# Autodesk Inventor assembly: ASY ДМФ 0100 Барабан v2.1
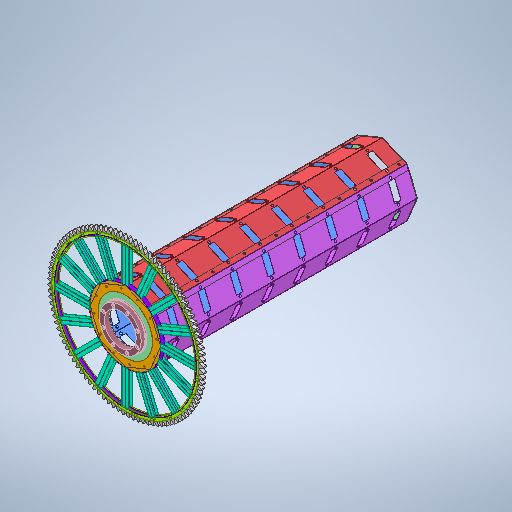
[picture p0: Inventor's stored thumbnail of the model, 512x512]
Saved by Autodesk Inventor 2025 (Build 290162010, 162A)
## iProperties
Created: 2024-04-28
Part Number: ASY ДМФ 0100 Барабан v2.1
Document SubType Name: Assembly
Designer: pokla
Author: pokla
## Documents named in this file (20)
- C:\Users\pokla\Documents\Inventor\ДФО\ДМФ\DMF-Disk-Micro-Filter\Барабан v2.1\ASY ДМФ 0100 Барабан v2.1.iam
- C:\Users\pokla\Documents\Inventor\ДФО\ДМФ\DMF-Disk-Micro-Filter\Барабан v2.1\DMF 01 21 Барабан торец НОС v2.1.ipt
- C:\Users\pokla\Documents\Inventor\ДФО\ДМФ\DMF-Disk-Micro-Filter\Барабан v2.1\DMF 01 13 Барабан Лист лев брт v2.1.ipt
- C:\Users\pokla\Documents\Inventor\ДФО\ДМФ\DMF-Disk-Micro-Filter\Барабан v2.1\DMF 01 14 Барабан Лист прав брт v2.1.ipt
- C:\Users\pokla\Documents\Inventor\ДФО\ДМФ\DMF-Disk-Micro-Filter\Барабан v2.1\DMF 01 31 Барабан Опорное кольцо НОС v2.1.ipt
- C:\Users\pokla\Documents\Inventor\ДФО\ДМФ\DMF-Disk-Micro-Filter\Барабан v2.1\DMF 01 17 опора крышки v2.1.ipt
- C:\Users\pokla\Documents\Inventor\ДФО\ДМФ\DMF-Disk-Micro-Filter\Барабан v2.1\DMF 000 размеры v2.1.ipt
- C:\Users\pokla\Documents\Inventor\ДФО\ДМФ\DMF-Disk-Micro-Filter\Барабан v2.1\DMF 01 12 Барабан усилитель v2.1.ipt
- C:\Users\pokla\Documents\Inventor\ДФО\ДМФ\DMF-Disk-Micro-Filter\Барабан v2.1\ASY DMF 010 cap v2.1.iam
- C:\Users\pokla\Documents\Inventor\ДФО\ДМФ\DMF-Disk-Micro-Filter\Барабан v2.1\DMF 01 32 Барабан Опорное кольцо КОРМА v2.1.ipt
- C:\Users\pokla\Documents\Inventor\ДФО\ДМФ\DMF-Disk-Micro-Filter\Барабан v2.1\DMF 01 22 Барабан торец КОРМА v2.1.ipt
- C:\Users\pokla\Documents\Inventor\ДФО\ДМФ\DMF-Disk-Micro-Filter\Барабан v2.1\ASY DMF filter package v2.1.iam
- C:\Users\pokla\Documents\Inventor\ДФО\ДМФ\DMF-Disk-Micro-Filter\Барабан v2.1\DMF 01 21 cylinder butt end nose.ipt
- C:\Users\pokla\Documents\Inventor\ДФО\ДМФ\DMF-Disk-Micro-Filter\Барабан v2.1\DMF 2.1 01 42 Gear way 2.ipt
- C:\Users\pokla\Documents\Inventor\ДФО\ДМФ\DMF-Disk-Micro-Filter\Барабан v2.1\DMF 2.1 01 43 Gear rim 3.ipt
- C:\Users\pokla\Documents\Inventor\ДФО\ДМФ\DMF-Disk-Micro-Filter\Барабан v2.1\DMF 2.1 01 44 Gear rim 4.ipt
- C:\Users\pokla\Documents\Inventor\ДФО\ДМФ\DMF-Disk-Micro-Filter\Барабан v2.1\DMF 2.1 01 45 Gear ring 5.ipt
- C:\Users\pokla\Documents\Inventor\ДФО\ДМФ\DMF-Disk-Micro-Filter\Барабан v2.1\DMF 2.1 01 46 Gear axis wheel 6.ipt
- C:\Users\pokla\Documents\Inventor\ДФО\ДМФ\DMF-Disk-Micro-Filter\Барабан v2.1\DMF 01 13 Барабан усилитель v2.1.ipt
- C:\Users\pokla\Documents\Inventor\ДФО\ДМФ\DMF-Disk-Micro-Filter\шестерни 06.09.2025\DMF sector big gear 2.1.ipt
## Components (104 placed, 25 different names)
1. DMF 000 размеры v2.1.ipt:1 — Rigid:30
2. DMF 01 21 Барабан торец НОС v2.1.ipt:1 — Mate:15, Flush:8, Flush:9, Flush:10, Flush:11, Mate:16, Mate:17, Mate:19, Mate:21, Flush:15, Flush:16, Flush:17, Mate:23, Rigid:29, Rigid:30, Rigid:33
3. DMF 01 31 Барабан Опорное кольцо НОС v2.1.ipt:1 — Rigid:29
4. DMF 01 32 Барабан Опорное кольцо КОРМА v2.1.ipt:1 — Rigid:20
5. DMF 01 22 Барабан торец КОРМА v2.1.ipt:1 — Flush:12, Flush:13, Mate:18, Rigid:20
6. DMF 01 13 Барабан Лист лев брт v2.1.ipt:1 — Flush:10, Flush:11, Mate:16, Flush:13, Mate:18, Mate:20, Mate:29
7. DMF 01 14 Барабан Лист прав брт v2.1.ipt:1 — Flush:8, Flush:9, Mate:17, Flush:12, Mate:22, Mate:28
8. DMF 01 17 опора крышки v2.1.ipt:1 — Mate:21, Flush:15, Mate:22
9. DMF 01 17 опора крышки v2.1.ipt:2 — Mate:19, Mate:20, Mate:27
10. ASY DMF 010 cap v2.1.iam:1 [sub-assembly] — Flush:16, Flush:17, Mate:23, Mate:27
11. DMF 01 21 cylinder butt end nose.ipt:1 — Mate:28, Mate:29
12. DMF 2.1 01 45 Gear ring 5.ipt:1 — Rigid:22, Rigid:23, Rigid:31, Rigid:32, Rigid:33, Flush:18, Mate:33, Mate:34
13. DMF 2.1 01 46 Gear axis wheel 6.ipt:1 — Rigid:31
14. ASY DMF filter package v2.1.iam:1 [sub-assembly] — Mate:24, Mate:25
15. ASY DMF filter package v2.1.iam:2 [sub-assembly]
16. ASY DMF filter package v2.1.iam:3 [sub-assembly]
17. ASY DMF filter package v2.1.iam:4 [sub-assembly]
18. ASY DMF filter package v2.1.iam:5 [sub-assembly]
19. ASY DMF filter package v2.1.iam:6 [sub-assembly]
20. ASY DMF filter package v2.1.iam:7 [sub-assembly]
21. ASY DMF filter package v2.1.iam:8 [sub-assembly]
22. DMF 2.1 01 44 Gear rim 4.ipt:1 — Rigid:22
23. DMF 2.1 01 44 Gear rim 4:2
24. DMF 2.1 01 44 Gear rim 4:3
25. DMF 2.1 01 43 Gear rim 3.ipt:1 — Rigid:24
26. DMF 2.1 01 43 Gear rim 3.ipt:2 — Rigid:23, Rigid:24
27. DMF 2.1 01 43 Gear rim 3:3
28. DMF 2.1 01 43 Gear rim 3:4
29. DMF 2.1 01 43 Gear rim 3:5
30. DMF 2.1 01 43 Gear rim 3:6
31. DMF 2.1 01 43 Gear rim 3:7
32. DMF 2.1 01 43 Gear rim 3:8
33. DMF sector big gear 2.1.ipt:1 — Rigid:32
34. DMF sector big gear 2.1:2
35. DMF sector big gear 2.1:3
36. DMF sector big gear 2.1:4
37. DMF sector big gear 2.1:5
38. DMF sector big gear 2.1:6
39. DMF sector big gear 2.1:7
40. DMF sector big gear 2.1:8
41. DMF sector big gear 2.1:9
42. DMF sector big gear 2.1:10
43. DMF sector big gear 2.1:11
44. DMF sector big gear 2.1:12
45. DMF sector big gear 2.1:13
46. DMF sector big gear 2.1:14
47. DMF sector big gear 2.1:15
48. DMF sector big gear 2.1:16
49. DMF sector big gear 2.1:17
50. DMF sector big gear 2.1:18
51. DMF sector big gear 2.1:19
52. DMF sector big gear 2.1:20
53. DMF sector big gear 2.1:21
54. DMF sector big gear 2.1:22
55. DMF sector big gear 2.1:23
56. DMF sector big gear 2.1:24
57. DMF 01 12 Барабан усилитель v2.1.ipt:1 — Rigid:34
58. DMF 2.1 01 42 Gear way 2.ipt:1 — Mate:30, Mate:31, Mate:32, Mate:34
59. DMF 01 13 Барабан усилитель v2.1.ipt:1 — Mate:30, Mate:31, Mate:32, Rigid:34, Flush:18, Mate:33
60. DMF 01 12 Барабан усилитель v2.1:50
61. DMF 2.1 01 42 Gear way 2:2
62. ДМФ 01 13 Барабан усилитель v2.0:2
63. DMF 01 12 Барабан усилитель v2.1:51
64. DMF 2.1 01 42 Gear way 2:3
65. ДМФ 01 13 Барабан усилитель v2.0:3
66. DMF 01 12 Барабан усилитель v2.1:52
67. DMF 2.1 01 42 Gear way 2:4
68. ДМФ 01 13 Барабан усилитель v2.0:4
69. DMF 01 12 Барабан усилитель v2.1:53
70. DMF 2.1 01 42 Gear way 2:5
71. ДМФ 01 13 Барабан усилитель v2.0:5
72. DMF 01 12 Барабан усилитель v2.1:54
73. DMF 2.1 01 42 Gear way 2:6
74. ДМФ 01 13 Барабан усилитель v2.0:6
75. DMF 01 12 Барабан усилитель v2.1:55
76. DMF 2.1 01 42 Gear way 2:7
77. ДМФ 01 13 Барабан усилитель v2.0:7
78. DMF 01 12 Барабан усилитель v2.1:56
79. DMF 2.1 01 42 Gear way 2:8
80. ДМФ 01 13 Барабан усилитель v2.0:8
81. DMF 01 12 Барабан усилитель v2.1:57
82. DMF 2.1 01 42 Gear way 2:9
83. ДМФ 01 13 Барабан усилитель v2.0:9
84. DMF 01 12 Барабан усилитель v2.1:58
85. DMF 2.1 01 42 Gear way 2:10
86. ДМФ 01 13 Барабан усилитель v2.0:10
87. DMF 01 12 Барабан усилитель v2.1:59
88. DMF 2.1 01 42 Gear way 2:11
89. ДМФ 01 13 Барабан усилитель v2.0:11
90. DMF 01 12 Барабан усилитель v2.1:60
91. DMF 2.1 01 42 Gear way 2:12
92. ДМФ 01 13 Барабан усилитель v2.0:12
93. DMF 01 12 Барабан усилитель v2.1:61
94. DMF 2.1 01 42 Gear way 2:13
95. ДМФ 01 13 Барабан усилитель v2.0:13
96. DMF 01 12 Барабан усилитель v2.1:62
97. DMF 2.1 01 42 Gear way 2:14
98. ДМФ 01 13 Барабан усилитель v2.0:14
99. DMF 01 12 Барабан усилитель v2.1:63
100. DMF 2.1 01 42 Gear way 2:15
101. ДМФ 01 13 Барабан усилитель v2.0:15
102. DMF 01 12 Барабан усилитель v2.1:64
103. DMF 2.1 01 42 Gear way 2:16
104. ДМФ 01 13 Барабан усилитель v2.0:16
## Component patterns: (8 elements, first: ASY DMF filter package v2.1.iam:1), (3 elements, first: DMF 2.1 01 44 Gear rim 4.ipt:1), (4 elements, first: DMF 2.1 01 43 Gear rim 3.ipt:1 + DMF 2.1 01 43 Gear rim 3.ipt:2), (24 elements, first: DMF sector big gear 2.1.ipt:1), (16 elements, first: DMF 01 12 Барабан усилитель v2.1.ipt:1 + DMF 2.1 01 42 Gear way 2.ipt:1 + DMF 01 13 Барабан усилитель v2.1.ipt:1)
## Relationships (39: Mate 19, Flush 10, WeldJoint 10)
- Mate:15: DMF 01 21 Барабан торец НОС v2.1.ipt:1
- Flush:8: DMF 01 21 Барабан торец НОС v2.1.ipt:1 ↔ DMF 01 14 Барабан Лист прав брт v2.1.ipt:1
- Flush:9: DMF 01 21 Барабан торец НОС v2.1.ipt:1 ↔ DMF 01 14 Барабан Лист прав брт v2.1.ipt:1
- Flush:10: DMF 01 21 Барабан торец НОС v2.1.ipt:1 ↔ DMF 01 13 Барабан Лист лев брт v2.1.ipt:1
- Flush:11: DMF 01 21 Барабан торец НОС v2.1.ipt:1 ↔ DMF 01 13 Барабан Лист лев брт v2.1.ipt:1
- Mate:16: DMF 01 21 Барабан торец НОС v2.1.ipt:1 ↔ DMF 01 13 Барабан Лист лев брт v2.1.ipt:1
- Mate:17: DMF 01 21 Барабан торец НОС v2.1.ipt:1 ↔ DMF 01 14 Барабан Лист прав брт v2.1.ipt:1
- Flush:12: DMF 01 22 Барабан торец КОРМА v2.1.ipt:1 ↔ DMF 01 14 Барабан Лист прав брт v2.1.ipt:1
- Flush:13: DMF 01 22 Барабан торец КОРМА v2.1.ipt:1 ↔ DMF 01 13 Барабан Лист лев брт v2.1.ipt:1
- Mate:18: DMF 01 22 Барабан торец КОРМА v2.1.ipt:1 ↔ DMF 01 13 Барабан Лист лев брт v2.1.ipt:1
- Mate:19: DMF 01 21 Барабан торец НОС v2.1.ipt:1 ↔ DMF 01 17 опора крышки v2.1.ipt:2
- Mate:20: DMF 01 13 Барабан Лист лев брт v2.1.ipt:1 ↔ DMF 01 17 опора крышки v2.1.ipt:2
- Mate:21: DMF 01 21 Барабан торец НОС v2.1.ipt:1 ↔ DMF 01 17 опора крышки v2.1.ipt:1
- Flush:15 (-2 mm): DMF 01 21 Барабан торец НОС v2.1.ipt:1 ↔ DMF 01 17 опора крышки v2.1.ipt:1
- Mate:22: DMF 01 14 Барабан Лист прав брт v2.1.ipt:1 ↔ DMF 01 17 опора крышки v2.1.ipt:1
- Flush:16: DMF 01 21 Барабан торец НОС v2.1.ipt:1 ↔ ASY DMF 010 cap v2.1.iam:1
- Flush:17: DMF 01 21 Барабан торец НОС v2.1.ipt:1 ↔ ASY DMF 010 cap v2.1.iam:1
- Mate:23: DMF 01 21 Барабан торец НОС v2.1.ipt:1 ↔ ASY DMF 010 cap v2.1.iam:1
- Mate:24: ASY DMF filter package v2.1.iam:1
- Mate:25: ASY DMF filter package v2.1.iam:1
- Mate:27: DMF 01 17 опора крышки v2.1.ipt:2 ↔ ASY DMF 010 cap v2.1.iam:1
- Mate:28: DMF 01 14 Барабан Лист прав брт v2.1.ipt:1 ↔ DMF 01 21 cylinder butt end nose.ipt:1
- Mate:29: DMF 01 13 Барабан Лист лев брт v2.1.ipt:1 ↔ DMF 01 21 cylinder butt end nose.ipt:1
- Rigid:20 [WeldJoint]: DMF 01 32 Барабан Опорное кольцо КОРМА v2.1.ipt:1 ↔ DMF 01 22 Барабан торец КОРМА v2.1.ipt:1
- Rigid:22 [WeldJoint]: DMF 2.1 01 45 Gear ring 5.ipt:1 ↔ DMF 2.1 01 44 Gear rim 4.ipt:1
- Rigid:23 [WeldJoint]: DMF 2.1 01 45 Gear ring 5.ipt:1 ↔ DMF 2.1 01 43 Gear rim 3.ipt:2
- Rigid:24 [WeldJoint] (25 mm): DMF 2.1 01 43 Gear rim 3.ipt:1 ↔ DMF 2.1 01 43 Gear rim 3.ipt:2
- Rigid:29 [WeldJoint]: DMF 01 21 Барабан торец НОС v2.1.ipt:1 ↔ DMF 01 31 Барабан Опорное кольцо НОС v2.1.ipt:1
- Rigid:30 [WeldJoint]: DMF 000 размеры v2.1.ipt:1 ↔ DMF 01 21 Барабан торец НОС v2.1.ipt:1
- Rigid:31 [WeldJoint]: DMF 2.1 01 45 Gear ring 5.ipt:1 ↔ DMF 2.1 01 46 Gear axis wheel 6.ipt:1
- Rigid:32 [WeldJoint] (2.5 mm): DMF 2.1 01 45 Gear ring 5.ipt:1 ↔ DMF sector big gear 2.1.ipt:1
- Rigid:33 [WeldJoint]: DMF 01 21 Барабан торец НОС v2.1.ipt:1 ↔ DMF 2.1 01 45 Gear ring 5.ipt:1
- Mate:30: DMF 2.1 01 42 Gear way 2.ipt:1 ↔ DMF 01 13 Барабан усилитель v2.1.ipt:1
- Mate:31 (284 mm): DMF 2.1 01 42 Gear way 2.ipt:1 ↔ DMF 01 13 Барабан усилитель v2.1.ipt:1
- Mate:32: DMF 2.1 01 42 Gear way 2.ipt:1 ↔ DMF 01 13 Барабан усилитель v2.1.ipt:1
- Rigid:34 [WeldJoint] (29 mm): DMF 01 12 Барабан усилитель v2.1.ipt:1 ↔ DMF 01 13 Барабан усилитель v2.1.ipt:1
- Flush:18 (-2 mm): DMF 2.1 01 45 Gear ring 5.ipt:1 ↔ DMF 01 13 Барабан усилитель v2.1.ipt:1
- Mate:33: DMF 2.1 01 45 Gear ring 5.ipt:1 ↔ DMF 01 13 Барабан усилитель v2.1.ipt:1
- Mate:34 (282 mm): DMF 2.1 01 45 Gear ring 5.ipt:1 ↔ DMF 2.1 01 42 Gear way 2.ipt:1
